# Autodesk Inventor assembly: Pendulum Suspension Assembly
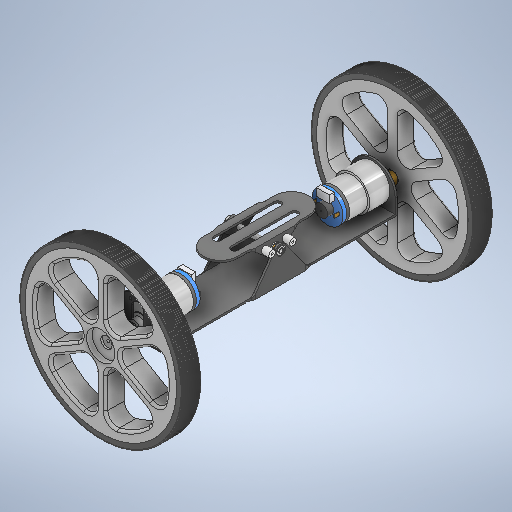
[picture p0: Inventor's stored thumbnail of the model, 512x512]
Saved by Autodesk Inventor 2025.2 (Build 292293000, 293)
## iProperties
Created: 2025-01-23
Part Number: Pendulum Suspension Assembly
Document SubType Name: Assembly
Designer: Matt Tidd
Author: Matt Tidd
## Documents named in this file (11)
- C:\Users\mtidd2\Desktop\H2A\CAD\Motors_and_Wheels\Pendulum Suspension\Pendulum Suspension Assembly.iam
- C:\Users\mtidd2\Desktop\H2A\CAD\Motors_and_Wheels\Pendulum Suspension\Pendulum Bottom Bracket.ipt
- C:\Users\mtidd2\Desktop\H2A\CAD\Motors_and_Wheels\Pendulum Suspension\Rotation Pin.ipt
- C:\Users\mtidd2\Desktop\H2A\CAD\Motors_and_Wheels\Pendulum Suspension\Rotation Bearing.ipt
- C:\Users\mtidd2\Desktop\H2A\CAD\Motors_and_Wheels\Pendulum Suspension\Rotation End Cap.ipt
- C:\Users\mtidd2\Desktop\H2A\CAD\Motors_and_Wheels\Pendulum Suspension\Pendulum Top Bracket.ipt
- C:\Users\mtidd2\Desktop\H2A\CAD\Motors_and_Wheels\520 DC Gear Motor.ipt
- C:\Users\mtidd2\Desktop\H2A\CAD\Motors_and_Wheels\Pendulum Suspension\Rotation Bumper.ipt
- C:\Users\mtidd2\Desktop\H2A\CAD\Motors_and_Wheels\520 DC Gear Motor Wheel Coupler.ipt
- C:\Users\mtidd2\Desktop\H2A\CAD\Motors_and_Wheels\Wheel Assembly\PLA Wheel Frame.ipt
- C:\Users\mtidd2\Desktop\H2A\CAD\Motors_and_Wheels\Wheel Assembly\TPU Tire.ipt
## Components (17 placed, 10 different names)
1. Pendulum Bottom Bracket:1 — Mate:2, Mate:6, Mate:9, Mate:10, Mate:11, Mate:12
2. Rotation Pin:1 — Mate:1
3. Rotation Bearing:1 — Mate:3, Mate:4
4. Rotation End Cap:1 — Mate:6
5. Rotation Bearing:2 — Mate:5
6. Rotation End Cap:2 — Mate:1, Mate:2, Mate:3
7. Pendulum Top Bracket:1 — Mate:4, Mate:5, Mate:7, Mate:8
8. 520 DC Gear Motor:1 — Mate:9, Mate:10, Mate:13
9. 520 DC Gear Motor:2 — Mate:11, Mate:12, Mate:16
10. Rotation Bumper:1 — Mate:7
11. Rotation Bumper:2 — Mate:8
12. 520 DC Gear Motor Wheel Coupler:1 — Mate:13, Mate:14, Mate:15
13. 520 DC Gear Motor Wheel Coupler:2 — Mate:16, Mate:17, Mate:18
14. PLA Wheel Frame:1 — Mate:14, Mate:15, Mate:21, Mate:22
15. PLA Wheel Frame:2 — Mate:17, Mate:18, Mate:19, Mate:20
16. TPU Tire:1 — Mate:21, Mate:22
17. TPU Tire:2 — Mate:19, Mate:20
## Relationships (22: Mate 22)
- Mate:1: Rotation Pin:1 ↔ Rotation End Cap:2
- Mate:2: Pendulum Bottom Bracket:1 ↔ Rotation End Cap:2
- Mate:3: Rotation Bearing:1 ↔ Rotation End Cap:2
- Mate:4: Rotation Bearing:1 ↔ Pendulum Top Bracket:1
- Mate:5: Rotation Bearing:2 ↔ Pendulum Top Bracket:1
- Mate:6: Pendulum Bottom Bracket:1 ↔ Rotation End Cap:1
- Mate:7: Pendulum Top Bracket:1 ↔ Rotation Bumper:1
- Mate:8: Pendulum Top Bracket:1 ↔ Rotation Bumper:2
- Mate:9: Pendulum Bottom Bracket:1 ↔ 520 DC Gear Motor:1
- Mate:10: Pendulum Bottom Bracket:1 ↔ 520 DC Gear Motor:1
- Mate:11: Pendulum Bottom Bracket:1 ↔ 520 DC Gear Motor:2
- Mate:12: Pendulum Bottom Bracket:1 ↔ 520 DC Gear Motor:2
- Mate:13: 520 DC Gear Motor:1 ↔ 520 DC Gear Motor Wheel Coupler:1
- Mate:14: 520 DC Gear Motor Wheel Coupler:1 ↔ PLA Wheel Frame:1
- Mate:15: 520 DC Gear Motor Wheel Coupler:1 ↔ PLA Wheel Frame:1
- Mate:16: 520 DC Gear Motor:2 ↔ 520 DC Gear Motor Wheel Coupler:2
- Mate:17: 520 DC Gear Motor Wheel Coupler:2 ↔ PLA Wheel Frame:2
- Mate:18: 520 DC Gear Motor Wheel Coupler:2 ↔ PLA Wheel Frame:2
- Mate:19: PLA Wheel Frame:2 ↔ TPU Tire:2
- Mate:20: PLA Wheel Frame:2 ↔ TPU Tire:2
- Mate:21: PLA Wheel Frame:1 ↔ TPU Tire:1
- Mate:22: PLA Wheel Frame:1 ↔ TPU Tire:1
